# Autodesk Inventor assembly: Cryostat
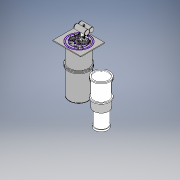
[picture p0: Inventor's stored thumbnail of the model, 180x180]
Saved by Autodesk Inventor 2018 (Build 220112000, 112)
## iProperties
Created: 2018-10-10
Part Number: Cryostat
Document SubType Name: Assembly
Designer: Admin
Author: Admin
## Documents named in this file (8)
- C:\Users\Admin\Documents\Cryostat\CAD\Cryostat.iam
- C:\Users\Admin\Documents\Cryostat\CAD\Top Plate V2.ipt
- C:\Users\Admin\Documents\Cryostat\CAD\External Models\CH40415 24JUL14 C.ipt
- C:\Users\Admin\Documents\Cryostat\CAD\Radiation Sheild 2K.ipt
- C:\Users\Admin\Documents\Cryostat\CAD\Radiation Sheild 55K bottom.ipt
- C:\Users\Admin\Documents\Cryostat\CAD\Radiation Sheild 55K.ipt
- C:\Users\Admin\Documents\Cryostat\CAD\vacuum jacket long.ipt
- C:\Users\Admin\Documents\Cryostat\CAD\vacuum jacket.ipt
## Components (7 placed, 7 different names)
1. Top Plate V2:1 — Mate:1, Mate:2, Mate:3, Mate:4, Mate:5, Mate:6
2. CH40415 24JUL14 C:1 — Mate:1, Mate:2, Mate:3
3. Radiation Sheild 2K:1
4. Radiation Sheild 55K bottom:1
5. Radiation Sheild 55K:1
6. vacuum jacket long:1 — Mate:7, Mate:8, Mate:9
7. vacuum jacket:1 — Mate:4, Mate:5, Mate:6, Mate:7, Mate:8, Mate:9
## Relationships (9: Mate 9)
- Mate:1: Top Plate V2:1 ↔ CH40415 24JUL14 C:1
- Mate:2: Top Plate V2:1 ↔ CH40415 24JUL14 C:1
- Mate:3: Top Plate V2:1 ↔ CH40415 24JUL14 C:1
- Mate:4: Top Plate V2:1 ↔ vacuum jacket:1
- Mate:5: Top Plate V2:1 ↔ vacuum jacket:1
- Mate:6: Top Plate V2:1 ↔ vacuum jacket:1
- Mate:7: vacuum jacket long:1 ↔ vacuum jacket:1
- Mate:8: vacuum jacket long:1 ↔ vacuum jacket:1
- Mate:9: vacuum jacket long:1 ↔ vacuum jacket:1
